# Autodesk Inventor assembly: EDM Machine+Shields
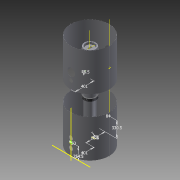
[picture p0: Inventor's stored thumbnail of the model, 180x180]
Saved by Autodesk Inventor 2015 (Build 190159000, 159)
## iProperties
Created: 2014-06-20
Part Number: EDM Machine+Shields
Document SubType Name: Assembly
Designer: Aki
Author: Aki
## Documents named in this file (16)
- C:\ColdMatter\CADFiles\EDM Machine\EDM Machine+Shields.iam
- C:\ColdMatter\CADFiles\EDM Machine\EDM Beamline\Chamber parts\hudson chamber actual size.ipt
- C:\ColdMatter\CADFiles\EDM Machine\EDM Inner Shield\Inner Shield.iam
- C:\ColdMatter\CADFiles\EDM Machine\EDM Beamline\Chamber parts\Centre nipple.iam
- C:\ColdMatter\CADFiles\EDM Machine\Electrical Feedthrough Collar\Electrical Feedthrough Collar.iam
- C:\ColdMatter\CADFiles\EDM Machine\Microwave Detection Region\Microwave Detection Region\Detection Region Chamber.iam
- C:\ColdMatter\CADFiles\EDM Machine\EDM Middle Shield\EDM Middle Shield Part 1.ipt
- C:\ColdMatter\CADFiles\EDM Machine\EDM Middle Shield\EDM Middle Shield Part 2.ipt
- C:\ColdMatter\CADFiles\EDM Machine\EDM Middle Shield\EDM Middle Shield Part 3.ipt
- C:\ColdMatter\CADFiles\EDM Machine\EDM Middle Shield\EDM Middle Shield Part 4.ipt
- C:\ColdMatter\CADFiles\EDM Machine\EDM Outer Shield\Lower Back Half.ipt
- C:\ColdMatter\CADFiles\EDM Machine\EDM Outer Shield\Lower Front Half.ipt
- C:\ColdMatter\CADFiles\EDM Machine\EDM Outer Shield\Upper Back Half.ipt
- C:\ColdMatter\CADFiles\EDM Machine\EDM Outer Shield\Upper Front Half.ipt
- C:\ColdMatter\CADFiles\EDM Machine\Microwave Detection Region\Probe Shield\Probe Shield Design.iam
- C:\ColdMatter\CADFiles\EDM Machine\Microwave Detection Region\Shield Support.iam
## Components (15 placed, 15 different names)
1. Inner Shield:1 [sub-assembly] — Mate:56, Mate:64
2. Centre nipple:1 [sub-assembly] — Mate:57, Mate:58, Mate:76, Mate:81
3. Electrical Feedthrough Collar:1 [sub-assembly] — Mate:65, Mate:76
4. Detection Region Chamber:1 [sub-assembly] — Mate:67, Mate:69, Mate:71, Mate:72, Mate:74, Mate:78
5. hudson chamber actual size:1 — Mate:55, Mate:56, Mate:57, Mate:79, Mate:80
6. EDM Middle Shield Part 1:1 — Mate:18, Mate:19, Mate:20, Mate:23, Mate:25, Mate:27, Mate:37
7. EDM Middle Shield Part 2:1 — Mate:18, Mate:19, Mate:21, Mate:22
8. EDM Middle Shield Part 3:1 — Mate:20, Mate:21, Mate:22, Mate:24
9. EDM Middle Shield Part 4:1 — Mate:23, Mate:24, Mate:25
10. Lower Back Half:1 — Mate:79, Mate:80, Mate:82, Mate:83
11. Lower Front Half:1 — Mate:81, Mate:82, Mate:83
12. Upper Back Half:1 — Mate:39, Mate:40, Mate:71, Mate:72
13. Upper Front Half:4 — Mate:37, Mate:39, Mate:40, Mate:73, Mate:77
14. Probe Shield Design:1 [sub-assembly] — Mate:73, Mate:74
15. Shield Support:1 [sub-assembly] — Mate:77, Mate:78
## Relationships (34: Mate 34)
- Mate:18: EDM Middle Shield Part 1:1 ↔ EDM Middle Shield Part 2:1
- Mate:19: EDM Middle Shield Part 1:1 ↔ EDM Middle Shield Part 2:1
- Mate:20: EDM Middle Shield Part 1:1 ↔ EDM Middle Shield Part 3:1
- Mate:21: EDM Middle Shield Part 2:1 ↔ EDM Middle Shield Part 3:1
- Mate:22: EDM Middle Shield Part 2:1 ↔ EDM Middle Shield Part 3:1
- Mate:23: EDM Middle Shield Part 1:1 ↔ EDM Middle Shield Part 4:1
- Mate:24: EDM Middle Shield Part 3:1 ↔ EDM Middle Shield Part 4:1
- Mate:25: EDM Middle Shield Part 1:1 ↔ EDM Middle Shield Part 4:1
- Mate:27: EDM Middle Shield Part 1:1
- Mate:37: EDM Middle Shield Part 1:1 ↔ Upper Front Half:4
- Mate:39: Upper Back Half:1 ↔ Upper Front Half:4
- Mate:40: Upper Back Half:1 ↔ Upper Front Half:4
- Mate:54
- Mate:55: hudson chamber actual size:1
- Mate:56: Inner Shield:1 ↔ hudson chamber actual size:1
- Mate:57: Centre nipple:1 ↔ hudson chamber actual size:1
- Mate:58: Centre nipple:1
- Mate:61
- Mate:64: Inner Shield:1
- Mate:65: Electrical Feedthrough Collar:1
- Mate:67: Detection Region Chamber:1
- Mate:69: Detection Region Chamber:1
- Mate:71: Detection Region Chamber:1 ↔ Upper Back Half:1
- Mate:72: Detection Region Chamber:1 ↔ Upper Back Half:1
- Mate:73: Upper Front Half:4 ↔ Probe Shield Design:1
- Mate:74: Detection Region Chamber:1 ↔ Probe Shield Design:1
- Mate:76: Centre nipple:1 ↔ Electrical Feedthrough Collar:1
- Mate:77: Upper Front Half:4 ↔ Shield Support:1
- Mate:78: Detection Region Chamber:1 ↔ Shield Support:1
- Mate:79: hudson chamber actual size:1 ↔ Lower Back Half:1
- Mate:80: hudson chamber actual size:1 ↔ Lower Back Half:1
- Mate:81: Centre nipple:1 ↔ Lower Front Half:1
- Mate:82: Lower Back Half:1 ↔ Lower Front Half:1
- Mate:83: Lower Back Half:1 ↔ Lower Front Half:1
